# Autodesk Inventor assembly: J005685
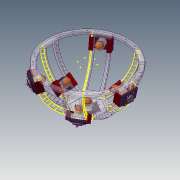
[picture p0: Inventor's stored thumbnail of the model, 180x180]
Saved by Autodesk Inventor 2015 SP1 (Build 190203100, 203)
## iProperties
Created: 2010-10-27
Part Number: J005685
Document SubType Name: Assembly
Designer: D Flickinger
Description: VR BALL BOWL ASSEMBLY
Vendor: HHMI: JRC - ID&F
Revision Number: 0
## Documents named in this file (11)
- C:\_WORKSPACE\DATA\COLLABORATION\SVOBODA LAB\MOUSE POSITIONING SYSTEMS\MCAD\BALL SETUP\MBS Bowl Assy.iam
- C:\_WORKSPACE\DATA\COLLABORATION\SVOBODA LAB\MOUSE POSITIONING SYSTEMS\MCAD\BALL SETUP\MBS AssemblyCanHolder.iam
- C:\_WORKSPACE\DATA\COLLABORATION\SVOBODA LAB\MOUSE POSITIONING SYSTEMS\MCAD\BALL SETUP\16 inch ball treadmill assembly.iam
- C:\_WORKSPACE\DATA\COLLABORATION\SVOBODA LAB\MOUSE POSITIONING SYSTEMS\MCAD\BALL SETUP\Ball_Rig\CanClamp.ipt
- C:\_WORKSPACE\DATA\COLLABORATION\SVOBODA LAB\MOUSE POSITIONING SYSTEMS\MCAD\BALL SETUP\Ball_Rig\ClamperPlate.ipt
- C:\_WORKSPACE\DATA\COLLABORATION\SVOBODA LAB\MOUSE POSITIONING SYSTEMS\MCAD\BALL SETUP\Ball_Rig\PingPongBall.ipt
- C:\_WORKSPACE\DATA\COLLABORATION\SVOBODA LAB\MOUSE POSITIONING SYSTEMS\MCAD\BALL SETUP\92185A194.ipt
- C:\_WORKSPACE\DATA\COLLABORATION\SVOBODA LAB\MOUSE POSITIONING SYSTEMS\MCAD\BALL SETUP\92185A203.ipt
- C:\_WORKSPACE\DATA\COLLABORATION\SVOBODA LAB\MOUSE POSITIONING SYSTEMS\MCAD\BALL SETUP\BallHolderTubeAirBall.ipt
- C:\_WORKSPACE\DATA\COLLABORATION\SVOBODA LAB\MOUSE POSITIONING SYSTEMS\MCAD\BALL SETUP\BottomCapAirBall.ipt
- C:\_WORKSPACE\DATA\COLLABORATION\SVOBODA LAB\MOUSE POSITIONING SYSTEMS\MCAD\BALL SETUP\50745K150.ipt
## Components (20 placed, 10 different names)
1. 16 inch ball treadmill assembly:1 [sub-assembly] — Mate:1, Mate:2, Mate:3, Mate:4, Mate:5, Mate:6, Mate:7, Mate:8, Mate:9, Mate:10, Mate:11, Mate:12, Mate:18, Flush:20, Angle:2, Mate:32, Mate:34, Mate:36
2. MBS AssemblyCanHolder:1 [sub-assembly] — Mate:3, Mate:4
3. MBS AssemblyCanHolder:2 [sub-assembly] — Mate:1, Mate:2
4. MBS AssemblyCanHolder:3 [sub-assembly] — Mate:11, Mate:12
5. MBS AssemblyCanHolder:4 [sub-assembly] — Mate:7, Mate:8
6. MBS AssemblyCanHolder:5 [sub-assembly] — Mate:5, Mate:6
7. MBS AssemblyCanHolder:6 [sub-assembly] — Mate:9, Mate:10
8. CanClamp:1 — Mate:37, Mate:38, Flush:21, Mate:39
9. ClamperPlate:1 — Mate:25, Mate:26, Mate:27, Mate:28, Mate:29, Mate:30, Mate:31, Mate:33, Mate:35
10. PingPongBall:1
11. 92185A194:1 — Mate:25, Mate:26
12. 92185A194:2 — Mate:31, Mate:32
13. 92185A194:3 — Mate:27, Mate:28
14. 92185A194:4 — Mate:29, Mate:30
15. 92185A194:5 — Mate:35, Mate:36
16. 92185A194:6 — Mate:33, Mate:34
17. 92185A203:1 — Mate:37, Mate:38
18. BallHolderTubeAirBall:1 — Flush:21, Mate:39, Mate:40, Mate:41
19. BottomCapAirBall:1 — Mate:40, Mate:41, Mate:42, Mate:43
20. 50745K150:1 — Mate:42, Mate:43
## Relationships (42: Mate 39, Flush 2, Angle 1)
- Mate:1: 16 inch ball treadmill assembly:1 ↔ MBS AssemblyCanHolder:2
- Mate:2: 16 inch ball treadmill assembly:1 ↔ MBS AssemblyCanHolder:2
- Mate:3: 16 inch ball treadmill assembly:1 ↔ MBS AssemblyCanHolder:1
- Mate:4: 16 inch ball treadmill assembly:1 ↔ MBS AssemblyCanHolder:1
- Mate:5: 16 inch ball treadmill assembly:1 ↔ MBS AssemblyCanHolder:5
- Mate:6: 16 inch ball treadmill assembly:1 ↔ MBS AssemblyCanHolder:5
- Mate:7: 16 inch ball treadmill assembly:1 ↔ MBS AssemblyCanHolder:4
- Mate:8: 16 inch ball treadmill assembly:1 ↔ MBS AssemblyCanHolder:4
- Mate:9: 16 inch ball treadmill assembly:1 ↔ MBS AssemblyCanHolder:6
- Mate:10: 16 inch ball treadmill assembly:1 ↔ MBS AssemblyCanHolder:6
- Mate:11: 16 inch ball treadmill assembly:1 ↔ MBS AssemblyCanHolder:3
- Mate:12: 16 inch ball treadmill assembly:1 ↔ MBS AssemblyCanHolder:3
- [Mate]: 16 inch ball treadmill assembly:1 ↔ ClamperPlate:1
- Mate:18: 16 inch ball treadmill assembly:1
- Flush:20 (-130.7084 mm): 16 inch ball treadmill assembly:1
- Angle:2 (60 deg): 16 inch ball treadmill assembly:1
- [Mate]: 16 inch ball treadmill assembly:1 ↔ ClamperPlate:1
- [Mate]: 16 inch ball treadmill assembly:1 ↔ ClamperPlate:1
- [Mate]: CanClamp:1 ↔ ClamperPlate:1
- [Mate]: CanClamp:1 ↔ ClamperPlate:1
- [Mate]: CanClamp:1 ↔ ClamperPlate:1
- [Mate]: CanClamp:1 ↔ ClamperPlate:1
- Mate:25: ClamperPlate:1 ↔ 92185A194:1
- Mate:26: ClamperPlate:1 ↔ 92185A194:1
- Mate:27: ClamperPlate:1 ↔ 92185A194:3
- Mate:28: ClamperPlate:1 ↔ 92185A194:3
- Mate:29: ClamperPlate:1 ↔ 92185A194:4
- Mate:30: ClamperPlate:1 ↔ 92185A194:4
- Mate:31: ClamperPlate:1 ↔ 92185A194:2
- Mate:32: 16 inch ball treadmill assembly:1 ↔ 92185A194:2
- Mate:33: ClamperPlate:1 ↔ 92185A194:6
- Mate:34: 16 inch ball treadmill assembly:1 ↔ 92185A194:6
- Mate:35: ClamperPlate:1 ↔ 92185A194:5
- Mate:36: 16 inch ball treadmill assembly:1 ↔ 92185A194:5
- Mate:37: CanClamp:1 ↔ 92185A203:1
- Mate:38: CanClamp:1 ↔ 92185A203:1
- Flush:21 (-5.08 mm): CanClamp:1 ↔ BallHolderTubeAirBall:1
- Mate:39: CanClamp:1 ↔ BallHolderTubeAirBall:1
- Mate:40 (1.27 mm): BallHolderTubeAirBall:1 ↔ BottomCapAirBall:1
- Mate:41: BallHolderTubeAirBall:1 ↔ BottomCapAirBall:1
- Mate:42: BottomCapAirBall:1 ↔ 50745K150:1
- Mate:43: BottomCapAirBall:1 ↔ 50745K150:1
